# Autodesk Inventor assembly: Rod turner
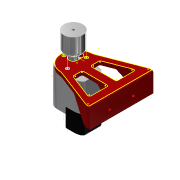
[picture p0: Inventor's stored thumbnail of the model, 180x180]
Saved by Autodesk Inventor 2013 (Build 170138000, 138)
## iProperties
Created: 2015-01-06
Part Number: Rod turner
Document SubType Name: Assembly
Designer: Nico
Author: Nico
## Documents named in this file (5)
- D:\Documents\Inventor\Fish Rod laquer Machine\Rod turner.iam
- D:\Documents\Inventor\Fish Rod laquer Machine\12V geared motor.ipt
- D:\Documents\Inventor\Fish Rod laquer Machine\motor holder.ipt
- D:\Documents\Inventor\Fish Rod laquer Machine\support shaft end.ipt
- D:\Documents\Inventor\Content Center Files\R2013\en-US\ANSI B18.6.5M(02)\ANSI B18.6.5M - 2.9x1 x 10(5).ipt
## Components (6 placed, 4 different names)
1. 12V geared motor:1 — Mate:1, Mate:2, Mate:3, Mate:4, Mate:5, Mate:9, Mate:10, Mate:11, Mate:12
2. support shaft end:1 — Mate:1, Mate:5
3. motor holder:1 — Mate:2, Mate:3, Mate:4, Flush:1, Flush:2, Flush:3, Mate:12, Mate:13
4. Cross Recessed Flat Countersunk Head Tapping Screw - Type B - Type I - Metric 2.9 x 1 x 10:1 — Mate:7, Flush:1
5. Cross Recessed Flat Countersunk Head Tapping Screw - Type B - Type I - Metric 2.9 x 1 x 10:2 — Mate:6, Flush:3
6. Cross Recessed Flat Countersunk Head Tapping Screw - Type B - Type I - Metric 2.9 x 1 x 10:3 — Mate:8, Flush:2
## Relationships (16: Mate 13, Flush 3)
- Mate:1: 12V geared motor:1 ↔ support shaft end:1
- Mate:2: 12V geared motor:1 ↔ motor holder:1
- Mate:3: 12V geared motor:1 ↔ motor holder:1
- Mate:4: 12V geared motor:1 ↔ motor holder:1
- Mate:5 (1 mm): 12V geared motor:1 ↔ support shaft end:1
- Mate:6: Cross Recessed Flat Countersunk Head Tapping Screw - Type B - Type I - Metric 2.9 x 1 x 10:2
- Mate:7: Cross Recessed Flat Countersunk Head Tapping Screw - Type B - Type I - Metric 2.9 x 1 x 10:1
- Mate:8: Cross Recessed Flat Countersunk Head Tapping Screw - Type B - Type I - Metric 2.9 x 1 x 10:3
- Mate:9: 12V geared motor:1
- Mate:10: 12V geared motor:1
- Mate:11: 12V geared motor:1
- Flush:1: motor holder:1 ↔ Cross Recessed Flat Countersunk Head Tapping Screw - Type B - Type I - Metric 2.9 x 1 x 10:1
- Flush:2: motor holder:1 ↔ Cross Recessed Flat Countersunk Head Tapping Screw - Type B - Type I - Metric 2.9 x 1 x 10:3
- Flush:3: motor holder:1 ↔ Cross Recessed Flat Countersunk Head Tapping Screw - Type B - Type I - Metric 2.9 x 1 x 10:2
- Mate:12: 12V geared motor:1 ↔ motor holder:1
- Mate:13: motor holder:1
